# Autodesk Inventor assembly: Subfloor
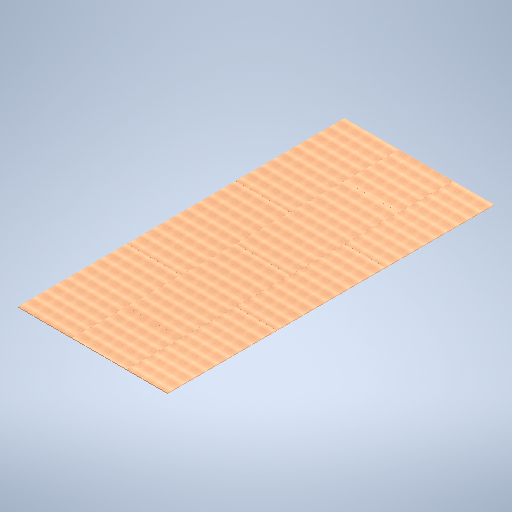
[picture p0: Inventor's stored thumbnail of the model, 512x512]
Saved by Autodesk Inventor 2025 (Build 290162010, 162A)
## iProperties
Created: 2024-09-19
Part Number: Subfloor
Document SubType Name: Assembly
Designer: Tom
Author: Tom
## Documents named in this file (4)
- C:\Users\Tom\Documents\Inventor\Mobility\Additional_Building\Subfloor.iam
- C:\Users\Tom\Documents\Inventor\Mobility\Additional_Building\OSB_For_Subfloor_With_Dimensions_96_x_48_Inches.ipt
- C:\Users\Tom\Documents\Inventor\Mobility\Additional_Building\OSB_For_Subfloor_With_Dimensions_48_x_48_Inches.ipt
- C:\Users\Tom\Documents\Inventor\Mobility\Additional_Building\OSB_For_Subfloor_With_Dimensions_96_x_36_Inches.ipt
## Components (10 placed, 3 different names)
1. OSB_For_Subfloor_With_Dimensions_96_x_48_Inches:1 — Mate:1, Flush:1, Mate:2
2. OSB_For_Subfloor_With_Dimensions_96_x_48_Inches:2
3. OSB_For_Subfloor_With_Dimensions_96_x_48_Inches:3
4. OSB_For_Subfloor_With_Dimensions_48_x_48_Inches:1 — Mate:1, Flush:1, Mate:3, Mate:4, Flush:2
5. OSB_For_Subfloor_With_Dimensions_48_x_48_Inches:2
6. OSB_For_Subfloor_With_Dimensions_96_x_48_Inches:4 — Mate:2, Mate:3
7. OSB_For_Subfloor_With_Dimensions_96_x_48_Inches:5
8. OSB_For_Subfloor_With_Dimensions_96_x_36_Inches:1 — Mate:4, Flush:2
9. OSB_For_Subfloor_With_Dimensions_96_x_36_Inches:2
10. OSB_For_Subfloor_With_Dimensions_96_x_36_Inches:3
## Component patterns: (3 elements, first: OSB_For_Subfloor_With_Dimensions_96_x_48_Inches:1), (2 elements, first: OSB_For_Subfloor_With_Dimensions_48_x_48_Inches:1), (2 elements, first: OSB_For_Subfloor_With_Dimensions_96_x_48_Inches:4), (3 elements, first: OSB_For_Subfloor_With_Dimensions_96_x_36_Inches:1)
## Relationships (6: Mate 4, Flush 2)
- Mate:1: OSB_For_Subfloor_With_Dimensions_96_x_48_Inches:1 ↔ OSB_For_Subfloor_With_Dimensions_48_x_48_Inches:1
- Flush:1: OSB_For_Subfloor_With_Dimensions_96_x_48_Inches:1 ↔ OSB_For_Subfloor_With_Dimensions_48_x_48_Inches:1
- Mate:2: OSB_For_Subfloor_With_Dimensions_96_x_48_Inches:1 ↔ OSB_For_Subfloor_With_Dimensions_96_x_48_Inches:4
- Mate:3: OSB_For_Subfloor_With_Dimensions_48_x_48_Inches:1 ↔ OSB_For_Subfloor_With_Dimensions_96_x_48_Inches:4
- Mate:4: OSB_For_Subfloor_With_Dimensions_48_x_48_Inches:1 ↔ OSB_For_Subfloor_With_Dimensions_96_x_36_Inches:1
- Flush:2: OSB_For_Subfloor_With_Dimensions_48_x_48_Inches:1 ↔ OSB_For_Subfloor_With_Dimensions_96_x_36_Inches:1
